# Autodesk Inventor assembly: Kartesischer_Roboter_Modul
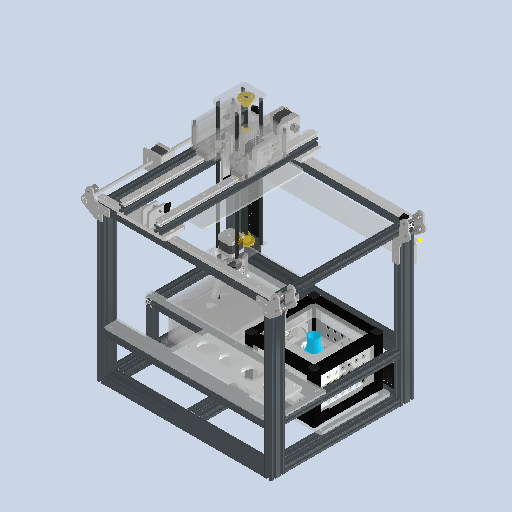
[picture p0: Inventor's stored thumbnail of the model, 512x512]
Saved by Autodesk Inventor 2022 (Build 260153000, 153)
## iProperties
Created: 2021-12-01
Part Number: Kartesischer_Roboter_Modul
Document SubType Name: Assembly
Designer: Fabijan_Sven
Author: Fabijan_Sven
## Documents named in this file (11)
- C:\Users\kaebi\OneDrive - mci4me.at\03_MCI Master\4.Semester_SS2022\Masterarbeit\Software\CAD_TeachingFactory\Kartesischer_Roboter_Modul.iam
- C:\Users\kaebi\OneDrive - mci4me.at\03_MCI Master\4.Semester_SS2022\Masterarbeit\Software\CAD_TeachingFactory\Gestell.iam
- C:\Users\kaebi\OneDrive - mci4me.at\03_MCI Master\4.Semester_SS2022\Masterarbeit\Software\CAD_TeachingFactory\Lager.iam
- C:\Users\kaebi\OneDrive - mci4me.at\03_MCI Master\4.Semester_SS2022\Masterarbeit\Software\CAD_TeachingFactory\ZB_Temperierstation.iam
- C:\Users\kaebi\OneDrive - mci4me.at\03_MCI Master\4.Semester_SS2022\Masterarbeit\Software\CAD_TeachingFactory\Kabelkanal_25x50_400.ipt
- C:\Users\kaebi\OneDrive - mci4me.at\03_MCI Master\4.Semester_SS2022\Masterarbeit\Software\CAD_TeachingFactory\Kabelkanal_25x50_477.ipt
- C:\Users\kaebi\OneDrive - mci4me.at\03_MCI Master\4.Semester_SS2022\Masterarbeit\Software\CAD_TeachingFactory\Ender.iam
- C:\Users\kaebi\OneDrive - mci4me.at\03_MCI Master\4.Semester_SS2022\Masterarbeit\Software\CAD_TeachingFactory\Waage.iam
- C:\Users\kaebi\OneDrive - mci4me.at\03_MCI Master\4.Semester_SS2022\Masterarbeit\Software\CAD_TeachingFactory\Steckerplatte1.ipt
- C:\Users\kaebi\OneDrive - mci4me.at\03_MCI Master\4.Semester_SS2022\Masterarbeit\Software\CAD_TeachingFactory\Steckerplatte_seit.ipt
- C:\Users\kaebi\OneDrive - mci4me.at\03_MCI Master\4.Semester_SS2022\Masterarbeit\Software\CAD_TeachingFactory\Steckerplatte_hint.ipt
## Components (10 placed, 10 different names)
1. Gestell:1 [sub-assembly] — Mate:1, Flush:2, Mate:2, Mate:5, Flush:3, Flush:4, Mate:8, Mate:9, Flush:6, Flush:7, Mate:10, Flush:8, Flush:14, Mate:17, Mate:18, Flush:15, Mate:19, Mate:20, Flush:16, Flush:17, Mate:24, Flush:18, Flush:19
2. Ender:1 [sub-assembly] — Mate:8, Mate:9, Flush:6
3. Lager:1 [sub-assembly] — Mate:1, Flush:2, Flush:8
4. ZB_Temperierstation:1 [sub-assembly] — Mate:2, Flush:7, Mate:10
5. Kabelkanal_25x37,5_330:1 — Mate:5, Flush:3, Flush:4
6. Kabelkanal_25x50_477:1 — Mate:18, Flush:15, Mate:19
7. Waage:1 [sub-assembly] — Flush:14, Mate:17
8. Steckerplatte1:1 — Mate:20, Flush:16, Flush:17, Mate:21, Mate:22, Mate:23
9. Steckerplatte_seit:1 — Mate:21, Mate:22, Mate:23
10. Steckerplatte_hint:1 — Mate:24, Flush:18, Flush:19
## Relationships (26: Mate 14, Flush 12)
- Mate:1: Gestell:1 ↔ Lager:1
- Flush:2: Gestell:1 ↔ Lager:1
- Mate:2: Gestell:1 ↔ ZB_Temperierstation:1
- Mate:5: Gestell:1 ↔ Kabelkanal_25x37,5_330:1
- Flush:3 (75 mm): Gestell:1 ↔ Kabelkanal_25x37,5_330:1
- Flush:4 (-2.5 mm): Gestell:1 ↔ Kabelkanal_25x37,5_330:1
- Mate:8: Gestell:1 ↔ Ender:1
- Mate:9: Gestell:1 ↔ Ender:1
- Flush:6: Gestell:1 ↔ Ender:1
- Flush:7: Gestell:1 ↔ ZB_Temperierstation:1
- Mate:10 (5 mm): Gestell:1 ↔ ZB_Temperierstation:1
- Flush:8: Gestell:1 ↔ Lager:1
- Flush:14: Gestell:1 ↔ Waage:1
- Mate:17: Gestell:1 ↔ Waage:1
- Mate:18: Gestell:1 ↔ Kabelkanal_25x50_477:1
- Flush:15: Gestell:1 ↔ Kabelkanal_25x50_477:1
- Mate:19 (190 mm): Gestell:1 ↔ Kabelkanal_25x50_477:1
- Mate:20: Gestell:1 ↔ Steckerplatte1:1
- Flush:16: Gestell:1 ↔ Steckerplatte1:1
- Flush:17: Gestell:1 ↔ Steckerplatte1:1
- Mate:21: Steckerplatte1:1 ↔ Steckerplatte_seit:1
- Mate:22: Steckerplatte1:1 ↔ Steckerplatte_seit:1
- Mate:23: Steckerplatte1:1 ↔ Steckerplatte_seit:1
- Mate:24: Gestell:1 ↔ Steckerplatte_hint:1
- Flush:18: Gestell:1 ↔ Steckerplatte_hint:1
- Flush:19: Gestell:1 ↔ Steckerplatte_hint:1
